# Autodesk Inventor assembly: CompactSlide
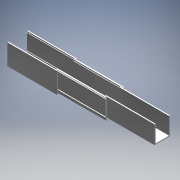
[picture p0: Inventor's stored thumbnail of the model, 180x180]
Saved by Autodesk Inventor 2019 (Build 230136000, 136)
## iProperties
Created: 2017-11-11
Part Number: CompactSlide
Document SubType Name: Assembly
Designer: User
Mass: 5226.12 g
Surface Area: 6805.11 cm^2
Volume: 1935.6 cm^3
Density: 2.7 g/cm^3
Author: User
## Documents named in this file (4)
- C:\Robotics\CAD\2017-18_CAD\Prototypes\CompactSlide.iam
- C:\Robotics\CAD\2017-18_CAD\Prototypes\CompactSlidePart1.ipt
- C:\Robotics\CAD\2017-18_CAD\Prototypes\CompactSlidePart2.ipt
- C:\Robotics\CAD\2017-18_CAD\Prototypes\CompactSlidePart3.ipt
## Components (3 placed, 3 different names)
1. CompactSlidePart1:1 — Mate:1, Mate:2, Mate:3
2. CompactSlidePart2:1 — Mate:1, Mate:2, Mate:3, Mate:4, Mate:5, Mate:6
3. CompactSlidePart3:1 — Mate:4, Mate:5, Mate:6
## Relationships (6: Mate 6)
- Mate:1: CompactSlidePart1:1 ↔ CompactSlidePart2:1
- Mate:2: CompactSlidePart1:1 ↔ CompactSlidePart2:1
- Mate:3 (-12.7 mm): CompactSlidePart1:1 ↔ CompactSlidePart2:1
- Mate:4 (1.5875 mm): CompactSlidePart2:1 ↔ CompactSlidePart3:1
- Mate:5 (1.5875 mm): CompactSlidePart2:1 ↔ CompactSlidePart3:1
- Mate:6 (-12.7 mm): CompactSlidePart2:1 ↔ CompactSlidePart3:1
